# Autodesk Inventor assembly: Fixture Assembly
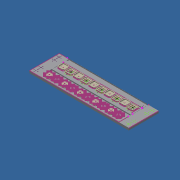
[picture p0: Inventor's stored thumbnail of the model, 180x180]
Saved by Autodesk Inventor 2016 (Build 200138000, 138)
## iProperties
Created: 2016-04-08
Part Number: Fixture Assembly
Document SubType Name: Assembly
Designer: Sam Clay
Author: Sam Clay
## Documents named in this file (6)
- Z:\enclosure\inventor\Fixture Assembly.iam
- Z:\enclosure\inventor\Fixture Base.ipt
- Z:\enclosure\inventor\Case Top.ipt
- Z:\enclosure\inventor\Case Bottom.ipt
- Z:\enclosure\inventor\Case Top Fixture.ipt
- Z:\enclosure\inventor\Case Bottom Fixture.ipt
## Components (21 placed, 5 different names)
1. Fixture Base:1 — Planar:6, Planar:7, Mate:4, Mate:5, Mate:6, Planar:8, Angle:1, Planar:9
2. Case Bottom:1 — Planar:6, Mate:6, Mate:7
3. Case Bottom:2
4. Case Bottom:3
5. Case Bottom:4
6. Case Bottom:5
7. Case Top:2 — Planar:7, Mate:4, Mate:5, Mate:7
8. Case Top:3
9. Case Top:4
10. Case Top:5
11. Case Top:6
12. Case Top Fixture:1 — Planar:9, Mate:8, Mate:9
13. Case Top Fixture:2
14. Case Top Fixture:3
15. Case Top Fixture:4
16. Case Top Fixture:5
17. Case Bottom Fixture:1 — Planar:8, Angle:1, Mate:8, Mate:9
18. Case Bottom Fixture:2
19. Case Bottom Fixture:3
20. Case Bottom Fixture:4
21. Case Bottom Fixture:5
## Component patterns: (5 elements, first: Case Bottom:1), (5 elements, first: Case Top:2), (5 elements, first: Case Top Fixture:1), (5 elements, first: Case Bottom Fixture:1)
## Relationships (11: Mate 6, PlanarJoint 4, Angle 1)
- Planar:6: Fixture Base:1 ↔ Case Bottom:1
- Planar:7: Fixture Base:1 ↔ Case Top:2
- Mate:4 (6.604 mm): Fixture Base:1 ↔ Case Top:2
- Mate:5 (6.604 mm): Fixture Base:1 ↔ Case Top:2
- Mate:6 (6.604 mm): Fixture Base:1 ↔ Case Bottom:1
- Mate:7 (6.604 mm): Case Bottom:1 ↔ Case Top:2
- Planar:8 (16.51 mm): Fixture Base:1 ↔ Case Bottom Fixture:1
- Angle:1 (0 deg): Fixture Base:1 ↔ Case Bottom Fixture:1
- Planar:9 (16.51 mm): Fixture Base:1 ↔ Case Top Fixture:1
- Mate:8 (-6.604 mm): Case Top Fixture:1 ↔ Case Bottom Fixture:1
- Mate:9: Case Top Fixture:1 ↔ Case Bottom Fixture:1
